# Autodesk Inventor assembly: N-2 rocket assembly1
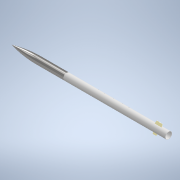
[picture p0: Inventor's stored thumbnail of the model, 180x180]
Saved by Autodesk Inventor 2020 (Build 240168000, 168)
## iProperties
Created: 2022-02-22
Part Number: N-2 rocket assembly1
Document SubType Name: Assembly
Designer: User
Author: User
## Documents named in this file (6)
- D:\N-2 rocket assembly1.iam
- D:\rocket parts airframe\body tube n-2.ipt
- D:\rocket parts airframe\nose cone n2.ipt
- D:\rocket parts airframe\extratube1.ipt
- D:\rocket parts airframe\extratube2.ipt
- D:\rocket parts airframe\fin set.ipt
## Components (8 placed, 5 different names)
1. body tube n-2:1 — Rigid:1, Mate:1, Mate:3, Rigid:2
2. nose cone n2:1 — Rotational:2
3. extratube1:1 — Rotational:2, Rigid:1
4. extratube1:2 — Mate:1, Mate:2, Mate:3, Rigid:2, Rigid:3
5. extratube2:1 — Mate:2, Rigid:4, Rigid:5
6. fin set:1 — Rigid:3
7. fin set:2 — Rigid:4
8. fin set:3 — Rigid:5
## Relationships (9: WeldJoint 5, Mate 3, RevoluteJoint 1)
- Rotational:2 [RevoluteJoint]: nose cone n2:1 ↔ extratube1:1
- Rigid:1 [WeldJoint]: body tube n-2:1 ↔ extratube1:1
- Mate:1: body tube n-2:1 ↔ extratube1:2
- Mate:2: extratube1:2 ↔ extratube2:1
- Mate:3: body tube n-2:1 ↔ extratube1:2
- Rigid:2 [WeldJoint]: body tube n-2:1 ↔ extratube1:2
- Rigid:3 [WeldJoint]: extratube1:2 ↔ fin set:1
- Rigid:4 [WeldJoint]: extratube2:1 ↔ fin set:2
- Rigid:5 [WeldJoint]: extratube2:1 ↔ fin set:3
